# Autodesk Inventor assembly: Assembly_Opentrons_Imagingunit_v2
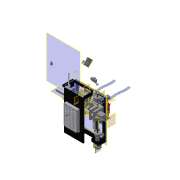
[picture p0: Inventor's stored thumbnail of the model, 180x180]
Saved by Autodesk Inventor 2019.4 (Build 234330000, 330)
## iProperties
Created: 2020-10-27
Part Number: Assembly_Opentrons_Imagingunit_v2
Document SubType Name: Assembly
Designer: diederichbenedict
Author: diederichbenedict
## Documents named in this file (17)
- C:\Users\diederichbenedict\Dropbox\Dokumente\Promotion\PROJECTS\OPENTRONS\INVENTOR\Assembly_Opentrons_Imagingunit_v2.iam
- C:\Users\diederichbenedict\Dropbox\Dokumente\Promotion\PROJECTS\OPENTRONS\INVENTOR\00_MTP_96-welplate.ipt
- C:\Users\diederichbenedict\Dropbox\Dokumente\Promotion\PROJECTS\OPENTRONS\INVENTOR\04_OPENTRONS_Microscope_wellplate_base.ipt
- C:\Users\diederichbenedict\Dropbox\Dokumente\Promotion\PROJECTS\OPENTRONS\INVENTOR\Assembly_opentrons_microscope_slide_y.iam
- C:\Users\diederichbenedict\Dropbox\Dokumente\Promotion\PROJECTS\OPENTRONS\INVENTOR\Assembly_opentrons_microscope_slide_y_base.iam
- C:\Users\diederichbenedict\Dropbox\Dokumente\Promotion\PROJECTS\OPENTRONS\INVENTOR\00_Endstop.ipt
- C:\Users\diederichbenedict\Dropbox\Dokumente\Promotion\PROJECTS\OPENTRONS\INVENTOR\Assembly_Opentrons_Autofocus_v1.iam
- C:\Users\diederichbenedict\Dropbox\Dokumente\Promotion\PROJECTS\OPENTRONS\INVENTOR\09_Opentrons_Microscope_Baseplate.ipt
- C:\Users\diederichbenedict\Dropbox\Dokumente\Promotion\PROJECTS\OPENTRONS\INVENTOR\00_MGN12 LINEAR GUIDE RAIL, CONFIGURABLE.ipt
- C:\Users\diederichbenedict\Dropbox\Dokumente\Promotion\PROJECTS\OPENTRONS\INVENTOR\00_MGN12H, LINEAR GUIDE BLOCK.ipt
- C:\Users\diederichbenedict\Dropbox\Dokumente\Promotion\PROJECTS\OPENTRONS\INVENTOR\00_spindel_slide.ipt
- C:\Users\diederichbenedict\Dropbox\Dokumente\Promotion\PROJECTS\OPENTRONS\INVENTOR\00_Thorlabs_Rod_200mm.ipt
- C:\Users\diederichbenedict\Dropbox\Dokumente\Promotion\PROJECTS\OPENTRONS\INVENTOR\15_Opentrons_Additional_Slide.ipt
- C:\Users\diederichbenedict\Dropbox\Dokumente\Promotion\PROJECTS\OPENTRONS\INVENTOR\16_Opentrons_Microscope_Slide_Bearing.ipt
- C:\Users\diederichbenedict\Dropbox\Dokumente\Promotion\PROJECTS\OPENTRONS\INVENTOR\Assembly_Opentrons_Autofocus_v2.iam
- C:\Users\diederichbenedict\Dropbox\Dokumente\Promotion\PROJECTS\OPENTRONS\INVENTOR\OPENTRONS_Autofocus_clutch_Nema.ipt
- C:\Users\diederichbenedict\Dropbox\Dokumente\Promotion\PROJECTS\OPENTRONS\INVENTOR\Assembly_Opentrons_Autofocus_Astigmatism_v0.iam
## Components (16 placed, 16 different names)
1. 00_Endstop:1
2. Assembly_opentrons_microscope_slide_y_base:1 [sub-assembly] — Mate:18, Angle:3, Mate:23, Flush:3, Flush:4, Mate:31, Flush:5, Flush:6, Flush:7
3. Assembly_opentrons_microscope_slide_y:1 [sub-assembly] — Insert:1, Angle:3, Mate:19, Mate:20, Flush:1, Flush:8, Flush:9, Mate:32
4. 09_Opentrons_Microscope_Baseplate:1 — Mate:31, Flush:5
5. 00_spindel_slide:1 — Insert:1, Mate:18
6. 00_MGN12H, LINEAR GUIDE BLOCK:1 — Mate:19, Mate:20, Flush:1, Mate:21, Mate:22
7. 00_MGN12 LINEAR GUIDE RAIL, CONFIGURABLE:2 — Mate:21, Mate:22, Mate:23
8. 00_MTP_96-welplate:1 — Flush:3, Flush:4, Mate:28, Mate:29, Mate:30
9. 04_OPENTRONS_Microscope_wellplate_base:1 — Mate:28, Mate:29, Mate:30
10. 15_Opentrons_Additional_Slide:1 — Flush:6, Flush:7, Insert:2, Angle:4
11. 00_Thorlabs_Rod_200mm:1 — Insert:2
12. 16_Opentrons_Microscope_Slide_Bearing:1 — Flush:8, Flush:9
13. Assembly_Opentrons_Autofocus_v1:1 [sub-assembly]
14. Assembly_Opentrons_Autofocus_v2:1 [sub-assembly] — Mate:32, Angle:4
15. OPENTRONS_Autofocus_clutch_Nema:1
16. Assembly_Opentrons_Autofocus_Astigmatism_v0:1 [sub-assembly]
## Relationships (23: Mate 11, Flush 8, Insert 2, Angle 2)
- Insert:1: Assembly_opentrons_microscope_slide_y:1 ↔ 00_spindel_slide:1
- Mate:18: Assembly_opentrons_microscope_slide_y_base:1 ↔ 00_spindel_slide:1
- Angle:3 (180 deg): Assembly_opentrons_microscope_slide_y_base:1 ↔ Assembly_opentrons_microscope_slide_y:1
- Mate:19: Assembly_opentrons_microscope_slide_y:1 ↔ 00_MGN12H, LINEAR GUIDE BLOCK:1
- Mate:20 (1 mm): Assembly_opentrons_microscope_slide_y:1 ↔ 00_MGN12H, LINEAR GUIDE BLOCK:1
- Flush:1 (5 mm): Assembly_opentrons_microscope_slide_y:1 ↔ 00_MGN12H, LINEAR GUIDE BLOCK:1
- Mate:21: 00_MGN12H, LINEAR GUIDE BLOCK:1 ↔ 00_MGN12 LINEAR GUIDE RAIL, CONFIGURABLE:2
- Mate:22: 00_MGN12H, LINEAR GUIDE BLOCK:1 ↔ 00_MGN12 LINEAR GUIDE RAIL, CONFIGURABLE:2
- Mate:23 (2 mm): Assembly_opentrons_microscope_slide_y_base:1 ↔ 00_MGN12 LINEAR GUIDE RAIL, CONFIGURABLE:2
- Flush:3 (75 mm): Assembly_opentrons_microscope_slide_y_base:1 ↔ 00_MTP_96-welplate:1
- Flush:4 (75 mm): Assembly_opentrons_microscope_slide_y_base:1 ↔ 00_MTP_96-welplate:1
- Mate:28: 00_MTP_96-welplate:1 ↔ 04_OPENTRONS_Microscope_wellplate_base:1
- Mate:29 (-2 mm): 00_MTP_96-welplate:1 ↔ 04_OPENTRONS_Microscope_wellplate_base:1
- Mate:30 (-2 mm): 00_MTP_96-welplate:1 ↔ 04_OPENTRONS_Microscope_wellplate_base:1
- Mate:31: Assembly_opentrons_microscope_slide_y_base:1 ↔ 09_Opentrons_Microscope_Baseplate:1
- Flush:5: Assembly_opentrons_microscope_slide_y_base:1 ↔ 09_Opentrons_Microscope_Baseplate:1
- Flush:6: Assembly_opentrons_microscope_slide_y_base:1 ↔ 15_Opentrons_Additional_Slide:1
- Flush:7: Assembly_opentrons_microscope_slide_y_base:1 ↔ 15_Opentrons_Additional_Slide:1
- Insert:2: 15_Opentrons_Additional_Slide:1 ↔ 00_Thorlabs_Rod_200mm:1
- Flush:8: Assembly_opentrons_microscope_slide_y:1 ↔ 16_Opentrons_Microscope_Slide_Bearing:1
- Flush:9: Assembly_opentrons_microscope_slide_y:1 ↔ 16_Opentrons_Microscope_Slide_Bearing:1
- Mate:32: Assembly_opentrons_microscope_slide_y:1 ↔ Assembly_Opentrons_Autofocus_v2:1
- Angle:4 (180 deg): 15_Opentrons_Additional_Slide:1 ↔ Assembly_Opentrons_Autofocus_v2:1
